# Autodesk Inventor assembly: switchlock
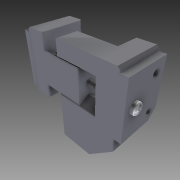
[picture p0: Inventor's stored thumbnail of the model, 180x180]
Saved by Autodesk Inventor 2015 (Build 190159000, 159)
## iProperties
Created: 2020-09-06
Part Number: switchlock
Document SubType Name: Assembly
Designer: penta
Author: penta
## Documents named in this file (7)
- C:\Users\penta\Documents\ArduinoBTAlarm\switchlock.iam
- C:\Users\penta\Documents\ArduinoBTAlarm\switchlock1l.ipt
- C:\Users\penta\Documents\ArduinoBTAlarm\switchlock1r.ipt
- C:\Users\penta\Documents\ArduinoBTAlarm\switchlock2l.ipt
- C:\Users\penta\Documents\ArduinoBTAlarm\switchlock2r.ipt
- C:\Users\penta\Documents\ArduinoBTAlarm\switchlock\디자인 액셀러레이터\볼트 연결1.iam
- C:\Users\penta\Documents\Inventor\Content Center Files\R2015\ko-KR\ISO 4036(2)\ISO 4036 - M2.5(2).ipt
## Components (6 placed, 6 different names)
1. switchlock1l:1 — 원통형:1
2. switchlock1r:1 — 원통형:1, 강체:3
3. switchlock2l:1 — 메이트:1, 메이트:2
4. switchlock2r:1
5. 볼트 연결:1 [sub-assembly] — 메이트:1, 메이트:2, 메이트:3
6. ISO 4036 M2.5:1 — 메이트:3, 강체:3
## Relationships (7: WeldJoint 3, Mate 3, CylindricalJoint 1)
- [WeldJoint]: switchlock1r:1 ↔ switchlock2r:1
- [WeldJoint]: switchlock1l:1 ↔ switchlock2l:1
- 원통형:1 [CylindricalJoint]: switchlock1l:1 ↔ switchlock1r:1
- 메이트:1 [Mate]: switchlock2l:1 ↔ 볼트 연결:1
- 메이트:2 [Mate]: switchlock2l:1 ↔ 볼트 연결:1
- 메이트:3 [Mate]: 볼트 연결:1 ↔ ISO 4036 M2.5:1
- 강체:3 [WeldJoint]: switchlock1r:1 ↔ ISO 4036 M2.5:1
## Named parameters: d = 8 mm
